# Autodesk Inventor assembly: fullAssembly1
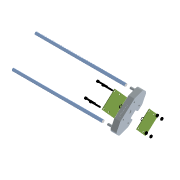
[picture p0: Inventor's stored thumbnail of the model, 180x180]
Saved by Autodesk Inventor 2020 (Build 240168000, 168)
## iProperties
Created: 2020-09-03
Part Number: fullAssembly1
Document SubType Name: Assembly
Designer: Admin
Author: Admin
## Documents named in this file (8)
- C:\PFE\Project_github\YFA-Project_python_interface\3D models\fullAssembly1.iam
- C:\PFE\Project_github\YFA-Project_python_interface\3D models\to_print_13_07\Housing_final.ipt
- C:\PFE\Project_github\YFA-Project_python_interface\3D models\to_print_11_08\7MMORING.ipt
- C:\PFE\Project_github\YFA-Project_python_interface\3D models\to_print_11_08\LED8.ipt
- C:\PFE\Project_github\YFA-Project_python_interface\3D models\to_print_11_08\TUBES.ipt
- C:\PFE\Project_github\YFA-Project_python_interface\3D models\to_print_11_08\SENSOR.ipt
- C:\PFE\Project_github\YFA-Project_python_interface\3D models\to_print_11_08\VIS.ipt
- C:\PFE\Project_github\YFA-Project_python_interface\3D models\to_print_11_08\NUT.ipt
## Components (15 placed, 7 different names)
1. Housing_final:1 — Mate:1, Mate:2, Mate:3, Mate:4, Mate:5, Mate:6, Mate:7, Mate:8
2. 7MMORING:1 — Mate:2
3. 7MMORING:2 — Mate:1
4. LED8:1 — Mate:3, Mate:4, Mate:13, Mate:14, Mate:15, Mate:16
5. TUBES:1 — Mate:5
6. TUBES:2 — Mate:6
7. SENSOR:1 — Mate:7, Mate:8, Mate:9, Mate:10, Mate:11, Mate:12
8. VIS:1 — Mate:12
9. VIS:2 — Mate:9
10. VIS:3 — Mate:11
11. VIS:4 — Mate:10
12. NUT:1 — Mate:13
13. NUT:2 — Mate:14
14. NUT:3 — Mate:16
15. NUT:4 — Mate:15
## Relationships (16: Mate 16)
- Mate:1: Housing_final:1 ↔ 7MMORING:2
- Mate:2: Housing_final:1 ↔ 7MMORING:1
- Mate:3: Housing_final:1 ↔ LED8:1
- Mate:4: Housing_final:1 ↔ LED8:1
- Mate:5: Housing_final:1 ↔ TUBES:1
- Mate:6: Housing_final:1 ↔ TUBES:2
- Mate:7: Housing_final:1 ↔ SENSOR:1
- Mate:8: Housing_final:1 ↔ SENSOR:1
- Mate:9: SENSOR:1 ↔ VIS:2
- Mate:10: SENSOR:1 ↔ VIS:4
- Mate:11: SENSOR:1 ↔ VIS:3
- Mate:12: SENSOR:1 ↔ VIS:1
- Mate:13: LED8:1 ↔ NUT:1
- Mate:14: LED8:1 ↔ NUT:2
- Mate:15: LED8:1 ↔ NUT:4
- Mate:16: LED8:1 ↔ NUT:3
